# Autodesk Inventor assembly: ASY TRM 020 star
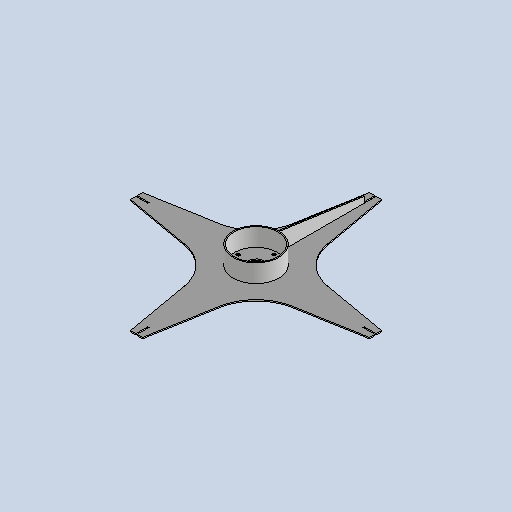
[picture p0: Inventor's stored thumbnail of the model, 512x512]
Saved by Autodesk Inventor 2025 (Build 290162010, 162A)
## iProperties
Created: 2024-09-08
Part Number: ASY TRM 020 star
Document SubType Name: Assembly
Designer: pokla
Author: pokla
## Documents named in this file (5)
- C:\Users\pokla\Documents\Inventor\BSH_Beshkino_bio_tank\ASY TRM 020 star.iam
- C:\Users\pokla\Documents\Inventor\BSH_Beshkino_bio_tank\TRM 029 coupling ring.ipt
- C:\Users\pokla\Documents\Inventor\BSH_Beshkino_bio_tank\TRM 030 star main.ipt
- C:\Users\pokla\Documents\Inventor\BSH_Beshkino_bio_tank\TRM 032 contrforce ring.ipt
- C:\Users\pokla\Documents\Inventor\BSH_Beshkino_bio_tank\TRM 030 star conrtforce plate.ipt
## Components (4 placed, 4 different names)
1. TRM 029 coupling ring:1
2. TRM 030 star main:1
3. TRM 032 contrforce ring:1
4. TRM 030 star conrtforce plate:1
## Relationships (3: WeldJoint 2, RevoluteJoint 1)
- [RevoluteJoint]: TRM 030 star main:1 ↔ TRM 032 contrforce ring:1
- [WeldJoint]: TRM 030 star main:1 ↔ TRM 030 star conrtforce plate:1
- [WeldJoint]: TRM 029 coupling ring:1 ↔ TRM 030 star main:1
